# Autodesk Inventor assembly: Rr.wing_assy
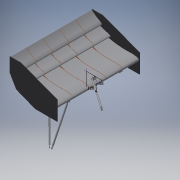
[picture p0: Inventor's stored thumbnail of the model, 180x180]
Saved by Autodesk Inventor 2018.2 (Build 222227000, 227)
## iProperties
Created: 2018-03-14
Part Number: Rr.wing_assy
Material: 一般
Document SubType Name: Assembly
Designer: ku_sk
Mass: 17392.7 g
Surface Area: 37058.8 cm^2
Volume: 16723.5 cm^3
Density: 1.04001 g/cm^3
Author: ku_sk
## Documents named in this file (17)
- C:\Users\ku_sk\Documents\Inventor\Aero\KS-15\Rr.wing\Rr.wing_assy.iam
- C:\Users\ku_sk\Documents\Inventor\Aero\KS-15\Rr.wing\parts\mainflap\mainflap.iam
- C:\Users\ku_sk\Documents\Inventor\Aero\KS-15\Rr.wing\parts\bracket.ipt
- C:\Users\ku_sk\Documents\Inventor\Aero\KS-15\Rr.wing\parts\subflap\subflap.iam
- C:\Users\ku_sk\Documents\Inventor\Aero\KS-15\Rr.wing\parts\endplate.ipt
- C:\Users\ku_sk\Documents\Inventor\Aero\KS-15\Rr.wing\parts\bracket2.ipt
- C:\Users\ku_sk\Documents\Inventor\Aero\KS-15\Rr.wing\parts\bracket3.ipt
- C:\Users\ku_sk\Documents\Inventor\Aero\KS-15\Rr.wing\parts\axis_r2.ipt
- C:\Users\ku_sk\Documents\Inventor\Aero\KS-15\Rr.wing\parts\axis_r1.ipt
- C:\Users\ku_sk\Documents\Inventor\Aero\KS-15\Rr.wing\parts\stay\stay1.iam
- C:\Users\ku_sk\Documents\Inventor\Aero\KS-15\Rr.wing\parts\stay\end\parts\Symmetry of POS_8ECBall.ipt
- C:\Users\ku_sk\Documents\Inventor\Aero\KS-15\Rr.wing\parts\stay\stay2.iam
- C:\Users\ku_sk\Documents\Inventor\Aero\KS-15\Rr.wing\parts\stay\stay3.iam
- C:\Users\ku_sk\Documents\Inventor\Aero\KS-15\Rr.wing\parts\stay\stay11.iam
- C:\Users\ku_sk\Documents\Inventor\Aero\KS-15\Rr.wing\parts\stay\stay21.iam
- C:\Users\ku_sk\Documents\Inventor\Aero\KS-15\Rr.wing\parts\stay\end\parts\Symmetry of POS_8ECBall1.ipt
- C:\Users\ku_sk\Documents\Inventor\Aero\KS-15\Rr.wing\parts\stay\stay31.iam
## Components (44 placed, 16 different names)
1. mainflap:1 [sub-assembly] — フラッシュ:1, メイト:1, 角度:1, メイト:2, メイト:3, メイト:4, メイト:5, メイト:6, メイト:7, メイト:9, メイト:10, メイト:12, メイト:13, メイト:18, メイト:19, メイト:24, メイト:25, メイト:57, メイト:61, メイト:72
2. mainflap:2 [sub-assembly] — メイト:8, メイト:9, メイト:10, メイト:20, メイト:21, メイト:22, メイト:67
3. mainflap:3 [sub-assembly] — メイト:11, メイト:12, メイト:13, メイト:14, メイト:16, メイト:17
4. mainflap:4 [sub-assembly] — メイト:23, メイト:24, メイト:25, メイト:56, メイト:70
5. mainflap:5 [sub-assembly] — メイト:15, メイト:18, メイト:19, メイト:60, メイト:65, メイト:71, メイト:77, メイト:78, フラッシュ:15
6. subflap:1 [sub-assembly] — メイト:26, メイト:27, メイト:28, メイト:73, メイト:74, フラッシュ:11
7. subflap:2 [sub-assembly] — メイト:29, メイト:30, メイト:31
8. subflap:3 [sub-assembly] — メイト:32, メイト:33, メイト:34, メイト:58, メイト:62
9. subflap:4 [sub-assembly] — メイト:35, メイト:36, メイト:37, メイト:39
10. subflap:5 [sub-assembly] — メイト:38, メイト:39, メイト:40
11. subflap:6 [sub-assembly] — メイト:41, メイト:42, メイト:43, メイト:75, メイト:76, フラッシュ:13
12. subflap:7 [sub-assembly] — メイト:44, メイト:45, メイト:46
13. subflap:8 [sub-assembly] — メイト:47, メイト:48, メイト:49, メイト:59, メイト:63
14. subflap:9 [sub-assembly] — メイト:50, メイト:51, メイト:52
15. subflap:10 [sub-assembly] — メイト:53, メイト:54, メイト:55
16. bracket:1 — メイト:20, メイト:21, メイト:22, メイト:23, メイト:26, メイト:27, メイト:28, メイト:29, メイト:30, メイト:31, メイト:41, メイト:42, メイト:43, メイト:44, メイト:45, メイト:46, メイト:83
17. bracket:2 — メイト:5, メイト:6, メイト:7, メイト:8, メイト:32, メイト:33, メイト:34, メイト:47, メイト:48, メイト:49
18. bracket:3 — メイト:2, メイト:3, メイト:4, メイト:11, メイト:35, メイト:36, メイト:37, メイト:50, メイト:51, メイト:52
19. bracket:4 — メイト:14, メイト:15, メイト:16, メイト:17, メイト:38, メイト:40, メイト:53, メイト:54, メイト:55, メイト:84
20. endplate:1 — メイト:56, メイト:57, メイト:58, メイト:59, 角度:2
21. endplate:2 — メイト:60, メイト:61, メイト:62, メイト:63
22. bracket2:3 — メイト:67, フラッシュ:4, フラッシュ:9, 角度:4, メイト:79, フラッシュ:16, メイト:85
23. bracket2:4 — メイト:65, フラッシュ:4, 角度:2, メイト:81, メイト:82, フラッシュ:17
24. bracket3:1 — メイト:70, フラッシュ:7, メイト:83, フラッシュ:16, メイト:86, メイト:87
25. bracket3:2 — メイト:71, フラッシュ:7, 角度:5, メイト:84, フラッシュ:17, メイト:88, メイト:89
26. bracket3:3 — メイト:72, フラッシュ:8, フラッシュ:9, 角度:4, 角度:5, メイト:90, メイト:91
27. axis_r2:1 — フラッシュ:12, メイト:76, フラッシュ:13
28. axis_r2:2 — フラッシュ:12, メイト:75
29. axis_r2:3 — フラッシュ:10, メイト:73
30. axis_r2:4 — フラッシュ:10, メイト:74, フラッシュ:11
31. axis_r1:1 — フラッシュ:14, メイト:78, フラッシュ:15
32. axis_r1:2 — フラッシュ:14, メイト:77
33. stay1:1 [sub-assembly] — 正接:1
34. stay11:1 [sub-assembly]
35. Symmetry of POS_8ECBall:1 — メイト:79, 正接:1, メイト:85
36. Symmetry of POS_8ECBall:2 — メイト:81, メイト:82
37. stay2:1 [sub-assembly] — 正接:2
38. stay21:1 [sub-assembly]
39. Symmetry of POS_8ECBall:3 — メイト:86, メイト:87, 正接:2
40. Symmetry of POS_8ECBall:4 — メイト:88, メイト:89
41. stay3:1 [sub-assembly] — 正接:3
42. stay31:1 [sub-assembly] — 正接:4
43. Symmetry of POS_8ECBall:5 — メイト:90, メイト:91, 正接:3
44. Symmetry of POS_8ECBall1:1 — 正接:4
## Relationships (107: Mate 86, Flush 13, Angle 4, Tangent 4)
- フラッシュ:1 [Flush]: mainflap:1
- メイト:1 [Mate]: mainflap:1
- 角度:1 [Angle] (15 deg): mainflap:1
- メイト:2 [Mate]: mainflap:1 ↔ bracket:3
- メイト:3 [Mate]: mainflap:1 ↔ bracket:3
- メイト:4 [Mate]: mainflap:1 ↔ bracket:3
- メイト:5 [Mate]: mainflap:1 ↔ bracket:2
- メイト:6 [Mate]: mainflap:1 ↔ bracket:2
- メイト:7 [Mate]: mainflap:1 ↔ bracket:2
- メイト:8 [Mate]: mainflap:2 ↔ bracket:2
- メイト:9 [Mate]: mainflap:1 ↔ mainflap:2
- メイト:10 [Mate]: mainflap:1 ↔ mainflap:2
- メイト:11 [Mate]: mainflap:3 ↔ bracket:3
- メイト:12 [Mate]: mainflap:1 ↔ mainflap:3
- メイト:13 [Mate]: mainflap:1 ↔ mainflap:3
- メイト:14 [Mate]: mainflap:3 ↔ bracket:4
- メイト:15 [Mate]: mainflap:5 ↔ bracket:4
- メイト:16 [Mate]: mainflap:3 ↔ bracket:4
- メイト:17 [Mate]: mainflap:3 ↔ bracket:4
- メイト:18 [Mate]: mainflap:1 ↔ mainflap:5
- メイト:19 [Mate]: mainflap:1 ↔ mainflap:5
- メイト:20 [Mate]: mainflap:2 ↔ bracket:1
- メイト:21 [Mate]: mainflap:2 ↔ bracket:1
- メイト:22 [Mate]: mainflap:2 ↔ bracket:1
- メイト:23 [Mate]: mainflap:4 ↔ bracket:1
- メイト:24 [Mate]: mainflap:1 ↔ mainflap:4
- メイト:25 [Mate]: mainflap:1 ↔ mainflap:4
- メイト:26 [Mate]: subflap:1 ↔ bracket:1
- メイト:27 [Mate]: subflap:1 ↔ bracket:1
- メイト:28 [Mate]: subflap:1 ↔ bracket:1
- メイト:29 [Mate]: subflap:2 ↔ bracket:1
- メイト:30 [Mate]: subflap:2 ↔ bracket:1
- メイト:31 [Mate]: subflap:2 ↔ bracket:1
- メイト:32 [Mate]: subflap:3 ↔ bracket:2
- メイト:33 [Mate]: subflap:3 ↔ bracket:2
- メイト:34 [Mate]: subflap:3 ↔ bracket:2
- メイト:35 [Mate]: subflap:4 ↔ bracket:3
- メイト:36 [Mate]: subflap:4 ↔ bracket:3
- メイト:37 [Mate]: subflap:4 ↔ bracket:3
- メイト:38 [Mate]: subflap:5 ↔ bracket:4
- メイト:39 [Mate]: subflap:4 ↔ subflap:5
- メイト:40 [Mate]: subflap:5 ↔ bracket:4
- メイト:41 [Mate]: subflap:6 ↔ bracket:1
- メイト:42 [Mate]: subflap:6 ↔ bracket:1
- メイト:43 [Mate]: subflap:6 ↔ bracket:1
- メイト:44 [Mate]: subflap:7 ↔ bracket:1
- メイト:45 [Mate]: subflap:7 ↔ bracket:1
- メイト:46 [Mate]: subflap:7 ↔ bracket:1
- メイト:47 [Mate]: subflap:8 ↔ bracket:2
- メイト:48 [Mate]: subflap:8 ↔ bracket:2
- メイト:49 [Mate]: subflap:8 ↔ bracket:2
- メイト:50 [Mate]: subflap:9 ↔ bracket:3
- メイト:51 [Mate]: subflap:9 ↔ bracket:3
- メイト:52 [Mate]: subflap:9 ↔ bracket:3
- メイト:53 [Mate]: subflap:10 ↔ bracket:4
- メイト:54 [Mate]: subflap:10 ↔ bracket:4
- メイト:55 [Mate]: subflap:10 ↔ bracket:4
- メイト:56 [Mate]: mainflap:4 ↔ endplate:1
- メイト:57 [Mate]: mainflap:1 ↔ endplate:1
- メイト:58 [Mate]: subflap:3 ↔ endplate:1
- メイト:59 [Mate]: subflap:8 ↔ endplate:1
- メイト:60 [Mate]: mainflap:5 ↔ endplate:2
- メイト:61 [Mate]: mainflap:1 ↔ endplate:2
- メイト:62 [Mate]: subflap:3 ↔ endplate:2
- メイト:63 [Mate]: subflap:8 ↔ endplate:2
- メイト:65 [Mate]: mainflap:5 ↔ bracket2:4
- メイト:67 [Mate]: mainflap:2 ↔ bracket2:3
- フラッシュ:4 [Flush]: bracket2:3 ↔ bracket2:4
- 角度:2 [Angle] (0 deg): endplate:1 ↔ bracket2:4
- メイト:70 [Mate]: mainflap:4 ↔ bracket3:1
- メイト:71 [Mate]: mainflap:5 ↔ bracket3:2
- フラッシュ:7 [Flush]: bracket3:1 ↔ bracket3:2
- メイト:72 [Mate]: mainflap:1 ↔ bracket3:3
- フラッシュ:8 [Flush]: bracket3:3
- フラッシュ:9 [Flush]: bracket2:3 ↔ bracket3:3
- 角度:4 [Angle] (0 deg): bracket2:3 ↔ bracket3:3
- 角度:5 [Angle] (0 deg): bracket3:2 ↔ bracket3:3
- フラッシュ:10 [Flush]: axis_r2:3 ↔ axis_r2:4
- メイト:73 [Mate]: subflap:1 ↔ axis_r2:3
- メイト:74 [Mate]: subflap:1 ↔ axis_r2:4
- フラッシュ:11 [Flush]: subflap:1 ↔ axis_r2:4
- フラッシュ:12 [Flush]: axis_r2:1 ↔ axis_r2:2
- メイト:75 [Mate]: subflap:6 ↔ axis_r2:2
- メイト:76 [Mate]: subflap:6 ↔ axis_r2:1
- フラッシュ:13 [Flush]: subflap:6 ↔ axis_r2:1
- フラッシュ:14 [Flush]: axis_r1:1 ↔ axis_r1:2
- メイト:77 [Mate]: mainflap:5 ↔ axis_r1:2
- メイト:78 [Mate]: mainflap:5 ↔ axis_r1:1
- フラッシュ:15 [Flush]: mainflap:5 ↔ axis_r1:1
- メイト:79 [Mate]: bracket2:3 ↔ Symmetry of POS_8ECBall:1
- メイト:81 [Mate]: bracket2:4 ↔ Symmetry of POS_8ECBall:2
- メイト:82 [Mate] (4.2 mm): bracket2:4 ↔ Symmetry of POS_8ECBall:2
- 正接:1 [Tangent]: stay1:1 ↔ Symmetry of POS_8ECBall:1
- メイト:83 [Mate] (4 mm): bracket:1 ↔ bracket3:1
- メイト:84 [Mate] (4 mm): bracket:4 ↔ bracket3:2
- フラッシュ:16 [Flush]: bracket2:3 ↔ bracket3:1
- フラッシュ:17 [Flush]: bracket2:4 ↔ bracket3:2
- メイト:85 [Mate] (4.2 mm): bracket2:3 ↔ Symmetry of POS_8ECBall:1
- メイト:86 [Mate]: bracket3:1 ↔ Symmetry of POS_8ECBall:3
- メイト:87 [Mate] (4.2 mm): bracket3:1 ↔ Symmetry of POS_8ECBall:3
- メイト:88 [Mate]: bracket3:2 ↔ Symmetry of POS_8ECBall:4
- メイト:89 [Mate] (4.2 mm): bracket3:2 ↔ Symmetry of POS_8ECBall:4
- 正接:2 [Tangent]: stay2:1 ↔ Symmetry of POS_8ECBall:3
- メイト:90 [Mate]: bracket3:3 ↔ Symmetry of POS_8ECBall:5
- メイト:91 [Mate] (5 mm): bracket3:3 ↔ Symmetry of POS_8ECBall:5
- 正接:3 [Tangent]: stay3:1 ↔ Symmetry of POS_8ECBall:5
- 正接:4 [Tangent]: stay31:1 ↔ Symmetry of POS_8ECBall1:1
